# Autodesk Inventor assembly: 200-40-BOGIE-CONNECTOR-REINFORCEMENT-01
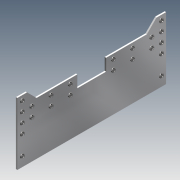
[picture p0: Inventor's stored thumbnail of the model, 180x180]
Saved by Autodesk Inventor 2018.2 (Build 222227000, 227)
## iProperties
Manager: feesmrt
Company: FRANCOR
Part Number: 200-40-BOGIE-CONNECTOR-REINFORCEMENT-01
Project: Rescue Robot
Cost Center: -
Material: Generisch
Document SubType Name: Assembly
Designer: feesmrt
Engineer: feesmrt
Authority: feesmrt
Description: Bogie Connector Verstärkung
Stock Number: 200-40-BOGIE-CONNECTOR-REINFORCEMENT-01
Subject: Rescue Robot
Author: feesmrt
Revision Number: 1
Title: Bogie Connector Verstärkung
## Documents named in this file (3)
- D:\Programmierung\FRANC0R\CAD\02-Rocker-Bogie-Robot\200-ROCKER-BOGIE\200-40-BOGIE-CONNECTOR\200-40-BOGIE-CONNECTOR-REINFORCEMENT-01.iam
- D:\Programmierung\FRANC0R\CAD\02-Rocker-Bogie-Robot\200-ROCKER-BOGIE\200-40-BOGIE-CONNECTOR\200-40-BOGIE-CONNECTOR-06.ipt
- D:\Programmierung\FRANC0R\CAD\02-Rocker-Bogie-Robot\200-ROCKER-BOGIE\200-40-BOGIE-CONNECTOR\200-40-BOGIE-CONNECTOR-REINFORCEMENT-02.iam
## Components (23 placed, 2 different names)
1. 200-40-BOGIE-CONNECTOR-06:1 — Passend:1, Passend:2, Winkel:1, Passend:3, Passend:4, Winkel:2, Passend:5, Passend:6, Winkel:3, Passend:7, Passend:8, Passend:9, Passend:10, Passend:11, Passend:12, Winkel:4, Winkel:5, Winkel:6
2. 200-40-BOGIE-CONNECTOR-REINFORCEMENT-02:5 [sub-assembly] — Passend:3, Passend:4, Winkel:2
3. 200-40-BOGIE-CONNECTOR-REINFORCEMENT-02:10 [sub-assembly] — Passend:8, Passend:12, Winkel:5
4. 200-40-BOGIE-CONNECTOR-REINFORCEMENT-02:1 [sub-assembly] — Passend:1, Passend:2, Winkel:1
5. 200-40-BOGIE-CONNECTOR-REINFORCEMENT-02:2 [sub-assembly]
6. 200-40-BOGIE-CONNECTOR-REINFORCEMENT-02:3 [sub-assembly]
7. 200-40-BOGIE-CONNECTOR-REINFORCEMENT-02:4 [sub-assembly]
8. 200-40-BOGIE-CONNECTOR-REINFORCEMENT-02:8 [sub-assembly] — Passend:5, Passend:6, Winkel:3
9. 200-40-BOGIE-CONNECTOR-REINFORCEMENT-02:12 [sub-assembly]
10. 200-40-BOGIE-CONNECTOR-REINFORCEMENT-02:13 [sub-assembly]
11. 200-40-BOGIE-CONNECTOR-REINFORCEMENT-02:14 [sub-assembly]
12. 200-40-BOGIE-CONNECTOR-REINFORCEMENT-02:15 [sub-assembly]
13. 200-40-BOGIE-CONNECTOR-REINFORCEMENT-02:16 [sub-assembly]
14. 200-40-BOGIE-CONNECTOR-REINFORCEMENT-02:9 [sub-assembly] — Passend:7, Passend:11, Winkel:4
15. 200-40-BOGIE-CONNECTOR-REINFORCEMENT-02:17 [sub-assembly]
16. 200-40-BOGIE-CONNECTOR-REINFORCEMENT-02:18 [sub-assembly]
17. 200-40-BOGIE-CONNECTOR-REINFORCEMENT-02:19 [sub-assembly]
18. 200-40-BOGIE-CONNECTOR-REINFORCEMENT-02:11 [sub-assembly] — Passend:9, Passend:10, Winkel:6
19. 200-40-BOGIE-CONNECTOR-REINFORCEMENT-02:20 [sub-assembly]
20. 200-40-BOGIE-CONNECTOR-REINFORCEMENT-02:21 [sub-assembly]
21. 200-40-BOGIE-CONNECTOR-REINFORCEMENT-02:22 [sub-assembly]
22. 200-40-BOGIE-CONNECTOR-REINFORCEMENT-02:23 [sub-assembly]
23. 200-40-BOGIE-CONNECTOR-REINFORCEMENT-02:24 [sub-assembly]
## Component patterns: (4 elements, first: 200-40-BOGIE-CONNECTOR-REINFORCEMENT-02:1), (6 elements, first: 200-40-BOGIE-CONNECTOR-REINFORCEMENT-02:8), (4 elements, first: 200-40-BOGIE-CONNECTOR-REINFORCEMENT-02:9), (6 elements, first: 200-40-BOGIE-CONNECTOR-REINFORCEMENT-02:11)
## Relationships (18: Mate 12, Angle 6)
- Passend:1 [Mate]: 200-40-BOGIE-CONNECTOR-06:1 ↔ 200-40-BOGIE-CONNECTOR-REINFORCEMENT-02:1
- Passend:2 [Mate]: 200-40-BOGIE-CONNECTOR-06:1 ↔ 200-40-BOGIE-CONNECTOR-REINFORCEMENT-02:1
- Winkel:1 [Angle] (0 deg): 200-40-BOGIE-CONNECTOR-06:1 ↔ 200-40-BOGIE-CONNECTOR-REINFORCEMENT-02:1
- Passend:3 [Mate]: 200-40-BOGIE-CONNECTOR-06:1 ↔ 200-40-BOGIE-CONNECTOR-REINFORCEMENT-02:5
- Passend:4 [Mate]: 200-40-BOGIE-CONNECTOR-06:1 ↔ 200-40-BOGIE-CONNECTOR-REINFORCEMENT-02:5
- Winkel:2 [Angle] (0 deg): 200-40-BOGIE-CONNECTOR-06:1 ↔ 200-40-BOGIE-CONNECTOR-REINFORCEMENT-02:5
- Passend:5 [Mate]: 200-40-BOGIE-CONNECTOR-06:1 ↔ 200-40-BOGIE-CONNECTOR-REINFORCEMENT-02:8
- Passend:6 [Mate]: 200-40-BOGIE-CONNECTOR-06:1 ↔ 200-40-BOGIE-CONNECTOR-REINFORCEMENT-02:8
- Winkel:3 [Angle] (0 deg): 200-40-BOGIE-CONNECTOR-06:1 ↔ 200-40-BOGIE-CONNECTOR-REINFORCEMENT-02:8
- Passend:7 [Mate]: 200-40-BOGIE-CONNECTOR-06:1 ↔ 200-40-BOGIE-CONNECTOR-REINFORCEMENT-02:9
- Passend:8 [Mate]: 200-40-BOGIE-CONNECTOR-06:1 ↔ 200-40-BOGIE-CONNECTOR-REINFORCEMENT-02:10
- Passend:9 [Mate]: 200-40-BOGIE-CONNECTOR-06:1 ↔ 200-40-BOGIE-CONNECTOR-REINFORCEMENT-02:11
- Passend:10 [Mate]: 200-40-BOGIE-CONNECTOR-06:1 ↔ 200-40-BOGIE-CONNECTOR-REINFORCEMENT-02:11
- Passend:11 [Mate]: 200-40-BOGIE-CONNECTOR-06:1 ↔ 200-40-BOGIE-CONNECTOR-REINFORCEMENT-02:9
- Passend:12 [Mate]: 200-40-BOGIE-CONNECTOR-06:1 ↔ 200-40-BOGIE-CONNECTOR-REINFORCEMENT-02:10
- Winkel:4 [Angle] (0 deg): 200-40-BOGIE-CONNECTOR-06:1 ↔ 200-40-BOGIE-CONNECTOR-REINFORCEMENT-02:9
- Winkel:5 [Angle] (0 deg): 200-40-BOGIE-CONNECTOR-06:1 ↔ 200-40-BOGIE-CONNECTOR-REINFORCEMENT-02:10
- Winkel:6 [Angle] (0 deg): 200-40-BOGIE-CONNECTOR-06:1 ↔ 200-40-BOGIE-CONNECTOR-REINFORCEMENT-02:11
